# Autodesk Inventor assembly: Battery
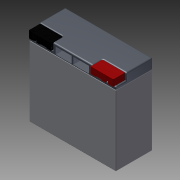
[picture p0: Inventor's stored thumbnail of the model, 180x180]
Saved by Autodesk Inventor 2015 (Build 190159000, 159)
## iProperties
Created: 2015-01-28
Part Number: Battery
Document SubType Name: Assembly
Designer: Andrew
Author: Autodesk
Title: C:\FRC_KOP_2015_Test\STEP\Electrical\ELEC_Battery_NP18-12B.iam.step
Description: 12V, 18AH, Deep Cycle
Creation Date: 2015-01-02
Sending System: Autodesk Inventor 2015
Preprocessor: ST-DEVELOPER v15.6
Author: Andrew
## Documents named in this file (5)
- C:\Users\pltwe4\Documents\recycling-rush\model\Battery.iam
- C:\Users\pltwe4\Documents\recycling-rush\model\Imported Components\ELEC_Battery_NP18-12B.iam\Electrical_Yuasa_NP18-12_Top.ipt
- C:\Users\pltwe4\Documents\recycling-rush\model\Imported Components\ELEC_Battery_NP18-12B.iam\Electrical_Yuasa_Np18-12_Middle.ipt
- C:\Users\pltwe4\Documents\recycling-rush\model\Battery Cap Negative.ipt
- C:\Users\pltwe4\Documents\recycling-rush\model\Battery Cap Positive.ipt
## Components (4 placed, 4 different names)
1. Electrical_Yuasa_NP18-12_Top:1 — Mate:1, Mate:2, Mate:3, Mate:4, Mate:5, Mate:6
2. Electrical_Yuasa_Np18-12_Middle:1
3. Battery Cap Negative:1 — Mate:4, Mate:5, Mate:6
4. Battery Cap Positive:1 — Mate:1, Mate:2, Mate:3
## Relationships (6: Mate 6)
- Mate:1: Electrical_Yuasa_NP18-12_Top:1 ↔ Battery Cap Positive:1
- Mate:2: Electrical_Yuasa_NP18-12_Top:1 ↔ Battery Cap Positive:1
- Mate:3: Electrical_Yuasa_NP18-12_Top:1 ↔ Battery Cap Positive:1
- Mate:4: Electrical_Yuasa_NP18-12_Top:1 ↔ Battery Cap Negative:1
- Mate:5: Electrical_Yuasa_NP18-12_Top:1 ↔ Battery Cap Negative:1
- Mate:6: Electrical_Yuasa_NP18-12_Top:1 ↔ Battery Cap Negative:1
